# Autodesk Inventor assembly: ASY МОО 001 отстойник осветлитель
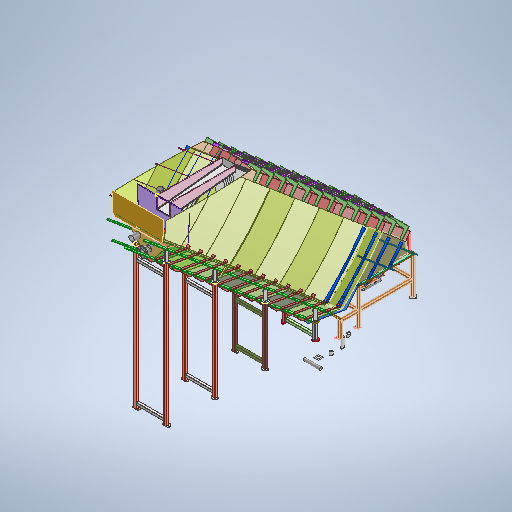
[picture p0: Inventor's stored thumbnail of the model, 512x512]
Saved by Autodesk Inventor 2025 (Build 290162010, 162A)
## iProperties
Created: 2024-04-28
Part Number: ASY МОО 001 отстойник осветлитель
Document SubType Name: Weldment
Designer: admin
Weld Material: Welded Aluminum-6061
Mass: 3.05393e+07 g
Surface Area: 3.06781e+06 cm^2
Volume: 2.84022e+07 cm^3
Density: 1.07525 g/cm^3
Author: admin
## Documents named in this file (67)
- C:\Users\user\YandexDisk\домашниий пк\Inventor\Manturovo\Manturovo_Se-clar\ASY MSC 001 отстойник осветлитель.iam
- C:\Users\user\YandexDisk\домашниий пк\Inventor\Manturovo\Manturovo_Se-clar\Рама основания\ASY MSC 090 base frame.iam
- C:\Users\user\YandexDisk\домашниий пк\Inventor\Manturovo\Manturovo_Se-clar\ASY MSC 080 roсket.iam
- C:\Users\user\YandexDisk\домашниий пк\Inventor\Manturovo\Manturovo_Se-clar\ASY MSC 010 cone.iam
- C:\Users\user\YandexDisk\домашниий пк\Inventor\Manturovo\Manturovo_Se-clar\ракета\МОО 064 ракета труба.ipt
- C:\Users\user\YandexDisk\домашниий пк\Inventor\Manturovo\Manturovo_Se-clar\MSC 000 DIM settler-clarifier.ipt
- C:\Users\user\YandexDisk\домашниий пк\Inventor\Manturovo\Manturovo_Se-clar\MSC 031 sheet lowerback.ipt
- C:\Users\user\YandexDisk\домашниий пк\Inventor\Manturovo\Manturovo_Se-clar\MSC 021 sheet left board hip.ipt
- C:\Users\user\YandexDisk\домашниий пк\Inventor\Manturovo\Manturovo_Se-clar\MSC 022 sheet right board hip.ipt
- C:\Users\user\YandexDisk\домашниий пк\Inventor\Manturovo\Manturovo_Se-clar\конус\MSC 071 ridge 1.ipt
- C:\Users\user\YandexDisk\домашниий пк\Inventor\Manturovo\Manturovo_Se-clar\конус\MSC 073 ridge 3.ipt
- C:\Users\user\YandexDisk\домашниий пк\Inventor\Manturovo\Manturovo_Se-clar\конус\MSC 074 face 1.ipt
- C:\Users\user\YandexDisk\домашниий пк\Inventor\Manturovo\Manturovo_Se-clar\Content Center Files\en-US\ISO 5251 B 3D\ISO 5251 Bends 3D without straight ends(90 deg) DN150 11 11.ipt
- C:\Users\user\YandexDisk\домашниий пк\Inventor\Manturovo\Manturovo_Se-clar\Content Center Files\en-US\DIN EN 1092-1 01 - PN 25\DIN EN 1092-1 Plate Flange for Welding Type 01 - PN 25 150 x 168.3.ipt
- C:\Users\user\YandexDisk\домашниий пк\Inventor\Manturovo\Manturovo_Se-clar\МОО 061 труба верх 1.ipt
- C:\Users\user\YandexDisk\домашниий пк\Inventor\Manturovo\Manturovo_Se-clar\МОО 062 труба верх 2.ipt
- C:\Users\user\YandexDisk\домашниий пк\Inventor\Manturovo\Manturovo_Se-clar\МОО 063 труба верх 3.ipt
- C:\Users\user\YandexDisk\домашниий пк\Inventor\Manturovo\Manturovo_Se-clar\Part1.ipt
- C:\Users\user\YandexDisk\домашниий пк\Inventor\Manturovo\Manturovo_Se-clar\MSC 0101 sheet gills.ipt
- C:\Users\user\YandexDisk\домашниий пк\Inventor\Manturovo\Manturovo_Se-clar\MSC 068 stringer lowerback.ipt
- C:\Users\user\YandexDisk\домашниий пк\Inventor\Manturovo\Manturovo_Se-clar\конус\MSC 072 ridge 2.ipt
- C:\Users\user\YandexDisk\домашниий пк\Inventor\Manturovo\Manturovo_Se-clar\MSC 075 face 2.ipt
- C:\Users\user\YandexDisk\домашниий пк\Inventor\Manturovo\Manturovo_Se-clar\MSC 076 face 3.ipt
- C:\Users\user\YandexDisk\домашниий пк\Inventor\Manturovo\Manturovo_Se-clar\MSC 077 face 4.ipt
- C:\Users\user\YandexDisk\домашниий пк\Inventor\Manturovo\Manturovo_Se-clar\MSC 110 revision hatch 1.ipt
- C:\Users\user\YandexDisk\домашниий пк\Inventor\Manturovo\Manturovo_Se-clar\MSC 035 ring.ipt
- C:\Users\user\YandexDisk\домашниий пк\Inventor\Manturovo\Manturovo_Se-clar\MSC 074 ridge 4.ipt
- C:\Users\user\YandexDisk\домашниий пк\Inventor\Manturovo\Manturovo_Se-clar\MSC 075 ridge 5.ipt
- C:\Users\user\YandexDisk\домашниий пк\Inventor\Manturovo\Manturovo_Se-clar\MSC 081 pillar 1.ipt
- C:\Users\user\YandexDisk\домашниий пк\Inventor\Manturovo\Manturovo_Se-clar\MSC 036 flange 500.ipt
- C:\Users\user\YandexDisk\домашниий пк\Inventor\Manturovo\Manturovo_Se-clar\MSC 037 flange cover 500.ipt
- C:\Users\user\YandexDisk\домашниий пк\Inventor\Manturovo\Manturovo_Se-clar\MSC 038 flange cover ring 500.ipt
- C:\Users\user\YandexDisk\домашниий пк\Inventor\Manturovo\Manturovo_Se-clar\MSC 039 flange cover plate 500.ipt
- C:\Users\user\YandexDisk\домашниий пк\Inventor\Manturovo\Manturovo_Se-clar\Рама основания\ASY MSC 120  base frame.iam
- C:\Users\user\YandexDisk\домашниий пк\Inventor\Manturovo\Manturovo_Se-clar\Рама основания\ASY MSC 121  base frame.iam
- C:\Users\user\YandexDisk\домашниий пк\Inventor\Manturovo\Manturovo_Se-clar\Чертеж для парам. рамы.ipt
- C:\Users\user\YandexDisk\домашниий пк\Inventor\Manturovo\Manturovo_Se-clar\ASY MSC 120.1  base frame.iam
- C:\Users\user\YandexDisk\домашниий пк\Inventor\Manturovo\Manturovo_Se-clar\ASY MSC 122  base frame.iam
- C:\Users\user\YandexDisk\домашниий пк\Inventor\Manturovo\Manturovo_Se-clar\ASY MSC 201 BACK.iam
- C:\Users\user\YandexDisk\домашниий пк\Inventor\Manturovo\Manturovo_Se-clar\ASY MSC 202 LEFT BOARD.iam
- C:\Users\user\YandexDisk\домашниий пк\Inventor\Manturovo\Manturovo_Se-clar\ASY MSC 203 RIGHT BOARD.iam
- C:\Users\user\YandexDisk\домашниий пк\Inventor\Manturovo\Manturovo_Se-clar\ASY MSC 204 BELLY.iam
- C:\Users\user\YandexDisk\домашниий пк\Inventor\Manturovo\Manturovo_Se-clar\MSC 063 stringer board #.ipt
- C:\Users\user\YandexDisk\домашниий пк\Inventor\Manturovo\Manturovo_Se-clar\MSC 064 stringer board ##.ipt
- C:\Users\user\YandexDisk\домашниий пк\Inventor\Manturovo\Manturovo_Se-clar\MSC 055 rib hip 2.ipt
- C:\Users\user\YandexDisk\домашниий пк\Inventor\Manturovo\Manturovo_Se-clar\MSC 054 rib hip 1.ipt
- C:\Users\user\YandexDisk\домашниий пк\Inventor\Manturovo\Manturovo_Se-clar\MSC 0102 sheet gills.ipt
- C:\Users\user\YandexDisk\домашниий пк\Inventor\Manturovo\Manturovo_Se-clar\MSC 078 creen pillar.iam
- C:\Users\user\YandexDisk\домашниий пк\Inventor\Manturovo\Manturovo_Se-clar\MSC 0202 sheet gills.ipt
- C:\Users\user\YandexDisk\домашниий пк\Inventor\Manturovo\Manturovo_Se-clar\MSC 0103 sheet gills.ipt
- C:\Users\user\YandexDisk\домашниий пк\Inventor\Manturovo\Manturovo_Se-clar\MSC 0203 sheet gills.ipt
- C:\Users\user\YandexDisk\домашниий пк\Inventor\Manturovo\Manturovo_Se-clar\MSC 0104 sheet gills.ipt
- C:\Users\user\YandexDisk\домашниий пк\Inventor\Manturovo\Manturovo_Se-clar\MSC 0204 sheet gills.ipt
- C:\Users\user\YandexDisk\домашниий пк\Inventor\Manturovo\Manturovo_Se-clar\MSC 0105 sheet gills.ipt
- C:\Users\user\YandexDisk\домашниий пк\Inventor\Manturovo\Manturovo_Se-clar\MSC 0205 sheet gills.ipt
- C:\Users\user\YandexDisk\домашниий пк\Inventor\Manturovo\Manturovo_Se-clar\MSC 0106 sheet gills.ipt
- C:\Users\user\YandexDisk\домашниий пк\Inventor\Manturovo\Manturovo_Se-clar\MSC 0206 sheet gills.ipt
- C:\Users\user\YandexDisk\домашниий пк\Inventor\Manturovo\Manturovo_Se-clar\MSC 0107 sheet gills.ipt
- C:\Users\user\YandexDisk\домашниий пк\Inventor\Manturovo\Manturovo_Se-clar\MSC 0207 sheet gills.ipt
- C:\Users\user\YandexDisk\домашниий пк\Inventor\Manturovo\Manturovo_Se-clar\MSC 079 creen pillar.ipt
- C:\Users\user\YandexDisk\домашниий пк\Inventor\Manturovo\Manturovo_Se-clar\ASY MSC 120 support.iam
- C:\Users\user\YandexDisk\домашниий пк\Inventor\Manturovo\Manturovo_Se-clar\конус\MSC 016 cone exit back.ipt
- C:\Users\user\YandexDisk\домашниий пк\Inventor\Manturovo\Manturovo_Se-clar\ракета\МОО 065 ракета труба 5.ipt
- C:\Users\user\YandexDisk\домашниий пк\Inventor\Manturovo\Manturovo_Se-clar\ракета\МОО 066 ракета труба 6.ipt
- C:\Users\user\YandexDisk\домашниий пк\Inventor\Manturovo\Manturovo_Se-clar\ракета\МОО 067 ракета труба 7.ipt
- C:\Users\user\YandexDisk\домашниий пк\Inventor\Manturovo\Manturovo_Se-clar\ракета\МОО 068 ракета труба 8.ipt
- C:\Users\user\YandexDisk\домашниий пк\Inventor\Manturovo\Manturovo_Se-clar\ракета\МОО 069 ракета труба 9.ipt
## Components (90 placed, 68 different names)
1. MSC 000 DIM settler-clarifier.ipt:1
2. MSC 001 DIM frame.ipt:1 — Flush:94, Mate:95, Mate:97, Mate:99, Mate:100
3. ASY MSC 120 support:1 [sub-assembly] — Mate:125, Cylindrical:6
4. ASY MSC 120 support:2 [sub-assembly] — Mate:129, Cylindrical:7
5. ASY MSC 120 support:3 [sub-assembly] — Mate:130, Cylindrical:8
6. ASY MSC 120 support:4 [sub-assembly] — Mate:131, Cylindrical:9
7. MSC 078 creen pillar:1 [sub-assembly]
8. ASY MSC 204 BELLY:1 [sub-assembly] — Mate:125, Mate:126, Mate:129, Mate:130, Mate:131, Mate:132, Mate:133
9. ASY MSC 203 RIGHT BOARD:1 [sub-assembly] — Tangent:17, Mate:126
10. ASY MSC 202 LEFT BOARD:1 [sub-assembly]
11. ASY MSC 201 BACK:1 [sub-assembly] — Mate:134
12. ASY MSC 122  base frame:2 [sub-assembly] — Flush:97, Mate:102, Cylindrical:9
13. ASY MSC 120.1  base frame:2 [sub-assembly] — Flush:96, Mate:100, Mate:101, Cylindrical:7
14. ASY MSC 121  base frame:1 [sub-assembly] — Mate:98, Flush:95, Mate:99, Cylindrical:8
15. ASY MSC 120  base frame:1 [sub-assembly] — Flush:93, Mate:97, Cylindrical:6
16. ASY MSC 080 roсket.iam:1 [sub-assembly] — Flush:23
17. MSC 016 cone exit back.ipt:1 — Rigid:208
18. ASY MSC 010 cone.iam:1 [sub-assembly] — Flush:22, Mate:16, Flush:28, Mate:65, Mate:78, Tangent:11, Flush:79, Mate:83, Flush:100
19. ASY MSC 090 base frame.iam:1 [sub-assembly] — Flush:19, Flush:21, Flush:82, Flush:100
20. МОО 064 ракета труба.ipt:1
21. MSC 031 sheet lowerback.ipt:1 — Mate:15, Mate:16, Tangent:10, Tangent:11, Tangent:12, Cylindrical:2, Rigid:185, Mate:134
22. MSC 021 sheet left board hip.ipt:1 — Flush:41, Mate:78
23. MSC 022 sheet right board hip.ipt:1 — Mate:30
24. MSC 071 ridge 1.ipt:1 — Mate:50, Flush:57, Mate:68, Flush:81, Flush:83, Mate:85
25. MSC 074 face 1.ipt:1 — Rigid:156, Rigid:157, Flush:62, Rigid:159, Mate:80, Mate:132, Mate:133
26. MSC 073 ridge 3.ipt:1 — Flush:57, Mate:68, Mate:77, Flush:78, Mate:81, Flush:80
27. МОО 061 труба верх 1.ipt:1 — Rigid:59, Rigid:159
28. ISO 5251 Bends 3D without straight ends(90 deg) DN150 11 11.ipt:1 — Rigid:59, Rotational:2
29. МОО 062 труба верх 2.ipt:1 — Rigid:132, Rigid:156
30. DIN EN 1092-1 Plate Flange for Welding Type 01 - PN 25 150 x 168.3.ipt:2 — Rigid:132
31. МОО 063 труба верх 3.ipt:1 — Rigid:157
32. Part1.ipt:1
33. MSC 068 stringer lowerback.ipt:1 — Mate:65, Tangent:10
34. MSC 072 ridge 2.ipt:1 — Flush:58, Mate:81, Flush:80, Flush:81, Flush:84
35. МОО 061 труба верх 1.ipt:2 — Rotational:2
36. MSC 075 face 2.ipt:1 — Flush:61
37. MSC 076 face 3.ipt:1 — Flush:76
38. MSC 077 face 4.ipt:1 — Mate:77, Flush:77, Flush:78, Mate:80
39. MSC 110 revision hatch 1:1 — Flush:82
40. MSC 068 stringer lowerback:2 — Mate:83, Tangent:12
41. MSC 035 ring:1 — Cylindrical:2, Rigid:185, Rigid:186
42. MSC 074 ridge 4:1 — Flush:83, Mate:85, Flush:84, Rigid:173
43. MSC 075 ridge 5:1 — Rigid:173
44. MSC 081 pillar 1:1
45. MSC 036 flange 500:1 — Rigid:175
46. MSC 036 flange 500:2 — Rigid:175, Rigid:176, Rigid:186
47. MSC 036 flange 500:3 — Rigid:176, Rigid:177, Mate:87
48. MSC 036 flange 500:4 — Rigid:177, Rotational:4
49. MSC 037 flange cover 500:1 — Rotational:4, Mate:87, Rigid:178, Mate:108
50. MSC 038 flange cover ring 500:1 — Rigid:178, Mate:109, Tangent:15
51. MSC 055 rib hip 2:2
52. MSC 063 stringer board #.ipt:2
53. MSC 064 stringer board ##.ipt:2
54. MSC 054 rib board hip 1:2
55. MSC 063 stringer board #.ipt:1
56. MSC 054 rib board hip 1:1
57. MSC 055 rib hip 2:1
58. MSC 064 stringer board ##.ipt:1
59. MSC 0102 sheet gills:1 — Rigid:197, Mate:124
60. MSC 0101 sheet gills.ipt:1
61. MSC 0202 sheet gills:1 — Rigid:197
62. MSC 0103 sheet gills:1 — Rigid:199, Mate:123, Mate:124
63. MSC 0203 sheet gills:1 — Rigid:199
64. MSC 0104 sheet gills:1 — Rigid:201, Mate:122, Mate:123
65. MSC 0204 sheet gills:1 — Rigid:201
66. MSC 0105 sheet gills:1 — Rigid:203, Mate:121, Mate:122
67. MSC 0205 sheet gills:1 — Rigid:203
68. MSC 0106 sheet gills:1 — Rigid:205, Mate:120, Mate:121
69. MSC 0206 sheet gills:1 — Rigid:205
70. MSC 0107 sheet gills:1 — Rigid:206, Mate:120
71. MSC 0207 sheet gills:1 — Rigid:206
72. MSC 079 creen pillar:2 — Tangent:17
73. МОО 064 ракета труба:2
74. МОО 065 ракета труба 5:1 — Rigid:209
75. МОО 066 ракета труба 6:1
76. МОО 067 ракета труба 7:1 — Rigid:208, Rigid:209
77. МОО 068 ракета труба 8:1
78. МОО 069 ракета труба 9:1
79. MSC 039 flange cover plate 500:1 — Mate:108, Mate:109, Tangent:15
80. MSC 039 flange cover plate 500:2
81. MSC 039 flange cover plate 500:3
82. MSC 039 flange cover plate 500:4
83. MSC 039 flange cover plate 500:5
84. MSC 039 flange cover plate 500:6
85. MSC 039 flange cover plate 500:7
86. MSC 039 flange cover plate 500:8
87. MSC 039 flange cover plate 500:9
88. MSC 039 flange cover plate 500:10
89. MSC 039 flange cover plate 500:11
90. MSC 039 flange cover plate 500:12
## Component patterns: (12 elements, first: MSC 039 flange cover plate 500:1)
## Relationships (109: Mate 42, Flush 27, WeldJoint 27, Tangent 5, CylindricalJoint 5, RevoluteJoint 2, Angle 1)
- [Flush]: ASY MSC 201 BACK:1
- Flush:19: ASY MSC 090 base frame.iam:1
- Flush:21: ASY MSC 090 base frame.iam:1
- Flush:22: ASY MSC 010 cone.iam:1
- Flush:23: ASY MSC 080 roсket.iam:1
- Mate:15: MSC 031 sheet lowerback.ipt:1
- Mate:16: ASY MSC 010 cone.iam:1 ↔ MSC 031 sheet lowerback.ipt:1
- Flush:28: ASY MSC 010 cone.iam:1
- [Flush]: ASY MSC 202 LEFT BOARD:1
- Flush:41: MSC 021 sheet left board hip.ipt:1
- Mate:30: MSC 022 sheet right board hip.ipt:1
- [Mate]: ASY MSC 202 LEFT BOARD:1 ↔ MSC 016 cone exit back.ipt:1
- Mate:50 (200 mm): MSC 071 ridge 1.ipt:1
- Rigid:59 [WeldJoint]: МОО 061 труба верх 1.ipt:1 ↔ ISO 5251 Bends 3D without straight ends(90 deg) DN150 11 11.ipt:1
- [Mate]: ASY MSC 203 RIGHT BOARD:1 ↔ MSC 016 cone exit back.ipt:1
- [Mate]: ASY MSC 203 RIGHT BOARD:1
- Rigid:132 [WeldJoint]: МОО 062 труба верх 2.ipt:1 ↔ DIN EN 1092-1 Plate Flange for Welding Type 01 - PN 25 150 x 168.3.ipt:2
- Mate:65: ASY MSC 010 cone.iam:1 ↔ MSC 068 stringer lowerback.ipt:1
- [Mate]: ASY MSC 201 BACK:1 ↔ MSC 068 stringer lowerback.ipt:1
- Tangent:10: MSC 031 sheet lowerback.ipt:1 ↔ MSC 068 stringer lowerback.ipt:1
- Flush:57: MSC 071 ridge 1.ipt:1 ↔ MSC 073 ridge 3.ipt:1
- Mate:68: MSC 071 ridge 1.ipt:1 ↔ MSC 073 ridge 3.ipt:1
- Flush:58 (200 mm): MSC 072 ridge 2.ipt:1
- Rotational:2 [RevoluteJoint]: ISO 5251 Bends 3D without straight ends(90 deg) DN150 11 11.ipt:1 ↔ МОО 061 труба верх 1.ipt:2
- Flush:61: MSC 075 face 2.ipt:1
- Rigid:156 [WeldJoint]: MSC 074 face 1.ipt:1 ↔ МОО 062 труба верх 2.ipt:1
- Rigid:157 [WeldJoint]: MSC 074 face 1.ipt:1 ↔ МОО 063 труба верх 3.ipt:1
- Flush:62: MSC 074 face 1.ipt:1
- Rigid:159 [WeldJoint] (-200 mm): MSC 074 face 1.ipt:1 ↔ МОО 061 труба верх 1.ipt:1
- Flush:76: MSC 076 face 3.ipt:1
- Mate:77: MSC 073 ridge 3.ipt:1 ↔ MSC 077 face 4.ipt:1
- Flush:77: MSC 077 face 4.ipt:1
- Flush:78: MSC 073 ridge 3.ipt:1 ↔ MSC 077 face 4.ipt:1
- Mate:78: ASY MSC 010 cone.iam:1 ↔ MSC 021 sheet left board hip.ipt:1
- Tangent:11 (22 mm): ASY MSC 010 cone.iam:1 ↔ MSC 031 sheet lowerback.ipt:1
- Flush:79: ASY MSC 010 cone.iam:1
- Mate:80: MSC 074 face 1.ipt:1 ↔ MSC 077 face 4.ipt:1
- Mate:81: MSC 073 ridge 3.ipt:1 ↔ MSC 072 ridge 2.ipt:1
- Flush:80: MSC 073 ridge 3.ipt:1 ↔ MSC 072 ridge 2.ipt:1
- Flush:81: MSC 071 ridge 1.ipt:1 ↔ MSC 072 ridge 2.ipt:1
- Flush:82: ASY MSC 090 base frame.iam:1 ↔ MSC 110 revision hatch 1:1
- Mate:83: ASY MSC 010 cone.iam:1 ↔ MSC 068 stringer lowerback:2
- [Mate]: ASY MSC 201 BACK:1 ↔ MSC 068 stringer lowerback:2
- Tangent:12: MSC 031 sheet lowerback.ipt:1 ↔ MSC 068 stringer lowerback:2
- Flush:83: MSC 071 ridge 1.ipt:1 ↔ MSC 074 ridge 4:1
- Mate:85: MSC 071 ridge 1.ipt:1 ↔ MSC 074 ridge 4:1
- Flush:84: MSC 072 ridge 2.ipt:1 ↔ MSC 074 ridge 4:1
- Rigid:173 [WeldJoint]: MSC 074 ridge 4:1 ↔ MSC 075 ridge 5:1
- Rigid:175 [WeldJoint]: MSC 036 flange 500:1 ↔ MSC 036 flange 500:2
- Rigid:176 [WeldJoint]: MSC 036 flange 500:2 ↔ MSC 036 flange 500:3
- Rigid:177 [WeldJoint]: MSC 036 flange 500:3 ↔ MSC 036 flange 500:4
- Cylindrical:2: MSC 031 sheet lowerback.ipt:1 ↔ MSC 035 ring:1
- Rotational:4 [RevoluteJoint]: MSC 036 flange 500:4 ↔ MSC 037 flange cover 500:1
- Mate:87: MSC 036 flange 500:3 ↔ MSC 037 flange cover 500:1
- Rigid:178 [WeldJoint]: MSC 037 flange cover 500:1 ↔ MSC 038 flange cover ring 500:1
- Flush:93 (-3 mm): ASY MSC 120  base frame:1
- [Mate]: ASY MSC 120  base frame:1
- Flush:94: MSC 001 DIM frame.ipt:1
- Mate:95: MSC 001 DIM frame.ipt:1
- Mate:97: MSC 001 DIM frame.ipt:1 ↔ ASY MSC 120  base frame:1
- Mate:98: ASY MSC 121  base frame:1
- Flush:95 (-3 mm): ASY MSC 121  base frame:1
- Mate:99: MSC 001 DIM frame.ipt:1 ↔ ASY MSC 121  base frame:1
- Flush:96 (-3 mm): ASY MSC 120.1  base frame:2
- Mate:100: MSC 001 DIM frame.ipt:1 ↔ ASY MSC 120.1  base frame:2
- Mate:101: ASY MSC 120.1  base frame:2
- Flush:97 (-3 mm): ASY MSC 122  base frame:2
- Mate:102: ASY MSC 122  base frame:2
- Rigid:185 [WeldJoint] (20 mm): MSC 031 sheet lowerback.ipt:1 ↔ MSC 035 ring:1
- Mate:108: MSC 037 flange cover 500:1 ↔ MSC 039 flange cover plate 500:1
- Mate:109: MSC 038 flange cover ring 500:1 ↔ MSC 039 flange cover plate 500:1
- Tangent:15: MSC 038 flange cover ring 500:1 ↔ MSC 039 flange cover plate 500:1
- Rigid:186 [WeldJoint]: MSC 035 ring:1 ↔ MSC 036 flange 500:2
- [WeldJoint] (2 mm): ASY MSC 203 RIGHT BOARD:1 ↔ MSC 064 stringer board ##.ipt:1
- [WeldJoint] (500 mm): ASY MSC 203 RIGHT BOARD:1 ↔ MSC 055 rib hip 2:1
- [WeldJoint] (500 mm): MSC 054 rib board hip 1:1 ↔ MSC 055 rib hip 2:1
- [WeldJoint] (2 mm): ASY MSC 202 LEFT BOARD:1 ↔ MSC 064 stringer board ##.ipt:2
- [WeldJoint] (500 mm): ASY MSC 202 LEFT BOARD:1 ↔ MSC 055 rib hip 2:2
- [WeldJoint] (500 mm): MSC 055 rib hip 2:2 ↔ MSC 054 rib board hip 1:2
- Rigid:197 [WeldJoint]: MSC 0102 sheet gills:1 ↔ MSC 0202 sheet gills:1
- Rigid:199 [WeldJoint]: MSC 0103 sheet gills:1 ↔ MSC 0203 sheet gills:1
- Rigid:201 [WeldJoint]: MSC 0104 sheet gills:1 ↔ MSC 0204 sheet gills:1
- Rigid:203 [WeldJoint]: MSC 0105 sheet gills:1 ↔ MSC 0205 sheet gills:1
- Rigid:205 [WeldJoint]: MSC 0106 sheet gills:1 ↔ MSC 0206 sheet gills:1
- Rigid:206 [WeldJoint]: MSC 0107 sheet gills:1 ↔ MSC 0207 sheet gills:1
- Mate:120 (50 mm): MSC 0106 sheet gills:1 ↔ MSC 0107 sheet gills:1
- Mate:121 (50 mm): MSC 0105 sheet gills:1 ↔ MSC 0106 sheet gills:1
- Mate:122 (50 mm): MSC 0104 sheet gills:1 ↔ MSC 0105 sheet gills:1
- Mate:123 (50 mm): MSC 0103 sheet gills:1 ↔ MSC 0104 sheet gills:1
- Mate:124 (50 mm): MSC 0102 sheet gills:1 ↔ MSC 0103 sheet gills:1
- Tangent:17: ASY MSC 203 RIGHT BOARD:1 ↔ MSC 079 creen pillar:2
- Mate:125: ASY MSC 120 support:1 ↔ ASY MSC 204 BELLY:1
- Mate:126: ASY MSC 204 BELLY:1 ↔ ASY MSC 203 RIGHT BOARD:1
- [Mate]: ASY MSC 204 BELLY:1 ↔ MSC 016 cone exit back.ipt:1
- [Angle] (0 deg): ASY MSC 204 BELLY:1 ↔ MSC 016 cone exit back.ipt:1
- Flush:100: ASY MSC 010 cone.iam:1 ↔ ASY MSC 090 base frame.iam:1
- Cylindrical:6: ASY MSC 120 support:1 ↔ ASY MSC 120  base frame:1
- Mate:129: ASY MSC 120 support:2 ↔ ASY MSC 204 BELLY:1
- Mate:130: ASY MSC 120 support:3 ↔ ASY MSC 204 BELLY:1
- Mate:131: ASY MSC 120 support:4 ↔ ASY MSC 204 BELLY:1
- Cylindrical:7: ASY MSC 120 support:2 ↔ ASY MSC 120.1  base frame:2
- Cylindrical:8: ASY MSC 120 support:3 ↔ ASY MSC 121  base frame:1
- Cylindrical:9: ASY MSC 120 support:4 ↔ ASY MSC 122  base frame:2
- Mate:132: ASY MSC 204 BELLY:1 ↔ MSC 074 face 1.ipt:1
- Mate:133: ASY MSC 204 BELLY:1 ↔ MSC 074 face 1.ipt:1
- Mate:134: ASY MSC 201 BACK:1 ↔ MSC 031 sheet lowerback.ipt:1
- [WeldJoint]: MSC 016 cone exit back.ipt:1 ↔ ASY MSC 010 cone.iam:1
- Rigid:208 [WeldJoint]: MSC 016 cone exit back.ipt:1 ↔ МОО 067 ракета труба 7:1
- Rigid:209 [WeldJoint]: МОО 065 ракета труба 5:1 ↔ МОО 067 ракета труба 7:1
## Named parameters: Бак_нахлест_фланца = 25 mm, Шаг_опор_по_баку = 2000 mm
